# Autodesk Inventor assembly: HUB BUILD PLATE
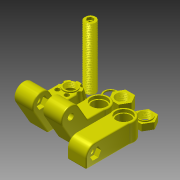
[picture p0: Inventor's stored thumbnail of the model, 180x180]
Saved by Autodesk Inventor 2013 (Build 170138000, 138)
## iProperties
Created: 2013-12-21
Part Number: HUB BUILD PLATE
Document SubType Name: Assembly
Designer: employee
Author: employee
## Documents named in this file (9)
- C:\Users\employee\Desktop\ConceptFORGE\ConceptFORGE\GUS Simpson\INVENTOR FILES\HUB BUILD PLATE.iam
- C:\Users\employee\Desktop\ConceptFORGE\ConceptFORGE\GUS Simpson\INVENTOR FILES\_BUILD PLATFORM.ipt
- C:\Users\employee\Desktop\ConceptFORGE\ConceptFORGE\GUS Simpson\INVENTOR FILES\HUB BOTTOM.ipt
- C:\Users\employee\Desktop\ConceptFORGE\ConceptFORGE\GUS Simpson\INVENTOR FILES\HUB SCREW.ipt
- C:\Users\employee\Desktop\ConceptFORGE\ConceptFORGE\GUS Simpson\INVENTOR FILES\HUB CENTER.ipt
- C:\Users\employee\Desktop\ConceptFORGE\ConceptFORGE\GUS Simpson\INVENTOR FILES\BOWDEN NUT.ipt
- C:\Users\employee\Desktop\ConceptFORGE\ConceptFORGE\GUS Simpson\INVENTOR FILES\LOCK NUT.ipt
- C:\Users\employee\Desktop\ConceptFORGE\ConceptFORGE\GUS Simpson\INVENTOR FILES\HUB TOP.ipt
- C:\Users\employee\Desktop\ConceptFORGE\ConceptFORGE\GUS Simpson\INVENTOR FILES\HUB WASHER.ipt
## Components (8 placed, 8 different names)
1. _BUILD PLATFORM:1 — Mate:1, Mate:2, Mate:3, Mate:4, Mate:5, Mate:6, Mate:7, Angle:1, Angle:2, Angle:3
2. HUB BOTTOM:1 — Mate:1, Angle:2
3. HUB SCREW:1 — Mate:2
4. HUB CENTER:1 — Mate:3, Angle:3
5. BOWDEN NUT:1 — Mate:4
6. LOCK NUT:1 — Mate:5
7. HUB TOP:1 — Mate:6, Angle:1
8. HUB WASHER:1 — Mate:7
## Relationships (10: Mate 7, Angle 3)
- Mate:1: _BUILD PLATFORM:1 ↔ HUB BOTTOM:1
- Mate:2: _BUILD PLATFORM:1 ↔ HUB SCREW:1
- Mate:3: _BUILD PLATFORM:1 ↔ HUB CENTER:1
- Mate:4: _BUILD PLATFORM:1 ↔ BOWDEN NUT:1
- Mate:5: _BUILD PLATFORM:1 ↔ LOCK NUT:1
- Mate:6: _BUILD PLATFORM:1 ↔ HUB TOP:1
- Mate:7: _BUILD PLATFORM:1 ↔ HUB WASHER:1
- Angle:1 (0 deg): _BUILD PLATFORM:1 ↔ HUB TOP:1
- Angle:2 (0 deg): _BUILD PLATFORM:1 ↔ HUB BOTTOM:1
- Angle:3 (0 deg): _BUILD PLATFORM:1 ↔ HUB CENTER:1
